# Autodesk Inventor assembly: SR-092-DPY(F,D-166-1)
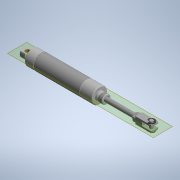
[picture p0: Inventor's stored thumbnail of the model, 180x180]
Saved by Autodesk Inventor 2020 (Build 240168000, 168)
## iProperties
Part Number: SR-092-DPY(F,D-166-1)
Catalog Web Link: www.cadenas.de
Description: Original Line Standard Air Cylinders-Standard Air Cylinders
Vendor: BIMBA
Document SubType Name: Assembly
Designer: partserver
Manufacturer: BIMBA
Mass: 56.1668 g
Surface Area: 355.51 cm^2
Volume: 56.1668 cm^3
Density: 1 g/cm^3
Category: PARTsolutions
Company: BIMBA
PSOL_IDENT_0: {$CADENAS_DATA\23d-libs\bimba\bimba_brand\bimba_imperial\bimba_full_line\original_line_cylinders\sta
PSOL_IDENT_1: ndard_air_cylinders\standard_air_cylinder_asmtab.prj},348 {VTYP=3D},{STYP=ASSTAB},{NB=SR-092-DPY(F,D
PSOL_IDENT_2: -166-1)},{LINA=SR-092-DPY(D-166-1)},{NN=Original Line Standard Air Cylinders},{DATE=19.01.2022 10:19
PSOL_IDENT_3: :38},{GEOMDATE=11.11.2021 07:31:43},{VERSION=},{LINEID=10},{WBVAR=STROKE,ACTING,MNT,DER,NR,BM,CO,OO,
PSOL_IDENT_4: VO,M,EE,EEL,K,Q,Y,G,T,HL,B,H,SER,SR,NT,W,STPT1,STPT2,STPT3,STPT4,MB,PB,PRC,TB,MN},{WBNUMERIC=STROKE,
PSOL_IDENT_5: EEL}  {NB=SR-092-DPY(F,D-166-1)},{LINA=SR-092-DPY(D-166-1)},{KT=DUMMY},{PN=SR-092-DPY},{PNC=SR-092-D
PSOL_IDENT_6: PY(F,D-166-1)},{PNA=(D-166-1)},{PNAHELP=(D-166-1)},{DASH=-},{BORE1=1.06250000},{BORE=1 1/16\" (09)},
PSOL_IDENT_7: {BOREPN=09},{STROKE=2.000},{STROKEALG=[0.011:50/0.001]},{STROKE1=2.000},{ACTING=D},{ACTINGALG= '' , '
PSOL_IDENT_8: Single Acting' , 'R' , 'Reverse Single Acting (R)' , 'D' , 'Double Acting (D)' },{ACTINGPN=D},{MNT=P
PSOL_IDENT_9: },{MNTALG= '' , 'Front Nose Mounting' , 'P' , 'Rear Pivot Mounting (P)' , 'X' , 'Universal Pivot Mou
PSOL_IDENT_10: nting or Double End Mounting (X)' , 'BF' , 'Front Block Mounting (BF)' , 'BR' , 'Rear Block Mounting
PSOL_IDENT_11: for Vertical Positioning (BR)' , 'BFT' , 'Front Block Trunnion Mounting (BFT)' , 'BRT' , 'Rear Bloc
PSOL_IDENT_12: k Trunnion Mounting (BRT)' },{TYPE=SR-},{MNTPN=P},{DER=},{DERALG= '' , 'N/A' },{NR=},{NRALG= '' , 'N
PSOL_IDENT_13: /A' },{NRPN=},{BM=},{BMALG= '' , 'N/A' },{BMPN=},{CO=},{COALG= '' , 'N/A' },{OO=},{OOALG= '', 'N/A'
PSOL_IDENT_14: },{OOPN=},{VO=Z},{VOALG= 'Z' , 'N/A' },{VOPN=},{OOVOPN=},{M=},{MALG= '', 'Without Magnet', 'M', 'Wit
PSOL_IDENT_15: h Magnet' },{EE=},{EEL=0.000},{EEMAX=48.0000},{EEALG= '', 'Without Extra Extension', 'EE', 'With Ext
PSOL_IDENT_16: ra Extension' },{EELALG=0},{EEPN=},{EEPN1=0.000},{K=},{KALG= '', 'Standard' , 'K' , 'Ports Rotated 9
PSOL_IDENT_17: 0deg K' },{KPN=},{Q=},{QALG= '' , 'N/A' },{QPN=},{Y=Y},{YALG= '' , 'Without Pivot Bushing' , 'Y' , '
PSOL_IDENT_18: With Pivot Bushing' },{YPN=Y},{YCON=Y},{F=},{FALG= '', 'Non-Coated (Standard)', 'F', 'Molycoated' },
PSOL_IDENT_19: {FPN=},{G=},{GPN=},{GPN99=},{T=},{TALG= '' , 'Standard -20° to 200°F (-29° to 95°C)' , 'N' , 'Low Te
PSOL_IDENT_20: mperature' , 'V' , 'High Temperature' },{NPN=},{VPN=},{HL=},{HLALG= '' , 'Without Low Pressure Hydra
PSOL_IDENT_21: ulic' , 'HL' , 'With Low Pressure Hydraulic' },{B=},{BALG= '', 'W/out Bumpers' , 'B' , 'W/ Bumpers'
PSOL_IDENT_22: },{BPN=},{H=},{HALG= '', 'N/A' },{HPN=},{SER=},{SERALG= '' , 'Without Spring Extend/Return' , 'JS' ,
PSOL_IDENT_23: 'With Spring Return' , 'JR' , 'With Spring Extend' },{SR=SR},{SRALG= 'C' , 'Standard Blackened Carb
PSOL_IDENT_24: on Steel' , 'SR' , 'Stainless Steel [SR]' },{SRPN=SR},{SRCON=1},{NT=},{NTPN=},{W=},{WALG= '' , 'With
PSOL_IDENT_25: out Wiper' , 'W' , 'With Wiper' },{WPN=},{E=},{EALG= '' , 'Standard Seals/Lube' , 'E' , 'Non-Lube Se
PSOL_IDENT_26: als/Lube' },{EPN=},{ST=},{STALG= '' , 'N/A' },{STPT1=},{STPT1ALG= '' , 'N/A' },{STPT2=},{STPT2ALG= ''
PSOL_IDENT_27: , 'N/A' },{STPT3=},{STPT3ALG= '' , 'N/A' },{STPT4=},{STPT4ALG= '' , 'N/A' },{STPN=},{MB=},{MBALG= ''
PSOL_IDENT_28: , 'N/A' },{MBPN=},{MBPNALL=},{MBPNALLREAR=},{PB=},{PBALG= '' , 'Without Pivot Bracket' , 'D-13498-A'
PSOL_IDENT_29: , 'D-13498-A' },{PBPN=},{PBPNALL=D-13498-A},{PRC=F,D-166-1},{PRCALG= '' , 'W/out Pivot Rod Clevis'
PSOL_IDENT_30: , 'F,D-166-1' , 'D-166-1 (front)' },{PRCPN=(F,D-166-1)},{PRCPNALL=D-166-1},{TB=},{TBALG= '' , 'N/A'
PSOL_IDENT_31: },{TBPN=},{TBPNALL=},{MN=},{MNALG= '' , 'Without Mounting Nut' , 'F,D-9' , 'D-9 (front)' , 'R,D-9' ,
PSOL_IDENT_32: 'D-9 (rear)', '2x,D-9' , 'D-9 (front & rear)' },{MNPN=},{MNCONF=},{MNCONR=},{TLEN=3.3185},{FRAC=8.8
PSOL_IDENT_33: 400},{RGCON=},{RGDACCON=R},{RHCON=P},{RHCON1=P},{RHCONON=1},{RHACCON=},{FNUTCON=0},{RNUTCON=0},{FNUT
PSOL_IDENT_34: PN=D-9},{RNUTPN=D-9},{FNUTTRANS=0.0000},{RNUTTRANS=0.0000},{VHOLECON=0},{A1=1.6250},{A1N=1.0000},{A1
PSOL_IDENT_35: P=1.6250},{A1B=1.8750},{A4=0.2525},{A4N=0.3750},{A4P=0.2525},{A5=0.0300},{A1H=1.5},{A1NH=0.6250},{A1
PSOL_IDENT_36: PH=1.5000},{A1BH=1.1250},{A1SH=1.1250},{A2H=0.2500},{A2NH=0.2500},{LENGTH=3.8400},{LENGTH1=3.8400},{
PSOL_IDENT_37: LENGTH2=4.1000},{MUL=2.0000},{MUL11=2.0000},{MUL22=5.12},{MUL33=3.1200},{MUL2=2.0000},{MUL211=2.0000
PSOL_IDENT_38: },{MUL222=2.5600},{MUL233=1.5600},{SSS=4.0000},{RGLEN=1.4025},{RHLEN=0.9990},{SSS1=3.0000},{A13=1.21
PSOL_IDENT_39: 90},{DIF=0.1200},{G5=0.7180},{ON=0},{SSADD=0.0000},{BADD=0.0000},{MADD=0.0000},{NVADD=0.0000},{TRACK
PSOL_IDENT_40: L=3.0285},{TRACKCON=D-78527},{TRIMCON=0},{TRIMCON1=0},{PINCON=},{FSPACE=0.7526},{SPACE=0.0911},{TEXT=
PSOL_IDENT_41: 0.1594},{S1=1.2500},{D1=1.1410},{D1N=1.1130},{D1B=1.1130},{D1P=1.1410},{FA=0.940},{RA=0.9400},{PPATH=
PSOL_IDENT_42: standard_air_cylinder_asmtpl.prj},{MATALGHTML=<b>Standard Original Line:</b><dl><dt>Rod:</dt><dd>- S
PSOL_IDENT_43: tainless Steel</dd><dd>&nbsp;&nbsp;(5/16 9/16 Bores)</dd><dd>- High Strength Carbon Steel</dd><dd>&n
PSOL_IDENT_44: bsp;&nbsp;(3/4 3 Bore)</dd><dd>- Stainless Steel</dd><dd>&nbsp;&nbsp;(X style DXP/DX/DXDE)</dd><dt>B
PSOL_IDENT_45: earings:</dt><dd>- Sintered Bronze</dd><dt>Body:</dt><dd>- 304 Stainless Steel</dd><dt>End Caps:</dt
PSOL_IDENT_46: ><dd>- Aluminum</dd><dt>Seals:</dt><dd>- Buna N</dd></dl>},{ASSCFGPRA=09DP},{MBPNA=},{MNPNA=},{PRCPN
PSOL_IDENT_47: A=(D-166-1)},{ASSOPTACC=STPT4},{A=5.84},{HADD=0.0000},{WFL=0.125},{QADD=0.000},{QADD1=0.250},{TEST=2
PSOL_IDENT_48: .0000},{MNTB=},{STDNUTF=0},{STDNUTR=0},{STRK2D=0},{X2D=2},{STROKESW=2.000},{EESW=0.000},{FCD=0},{BCD=
PSOL_IDENT_49: 0},{RCD=0},{CUSTADD=1.000},{FT=5/16-24 UNF-2A},{FT1=5/16-24 UNF-2A},{FT2=5/8-18 UNF-2A},{PORT=1/8 NP
PSOL_IDENT_50: T},{FT11=5/8-18 UNF-2A},{FT12=5/8-18 UNF-2A},{B1=}
NB: SR-092-DPY(F,D-166-1)
NN: Original Line Standard Air Cylinders
NT: Threaded (Standard)
NBSYN: $PNC.
LINA: SR-092-DPY(D-166-1)
CATALOG: Bimba Products
PN: SR-092-DPY
PNA: (D-166-1)
BORE: 1 1/16" (09)
STROKE: 2
ACTING: Double Acting (D)
MNT: Rear Pivot Mounting (P)
DER: N/A
NR: N/A
BM: N/A
CO: N/A
OO: N/A
VO: N/A
M: Without Magnet
EE: Without Extra Extension
EEL: 0
K: Standard
Q: N/A
Y: With Pivot Bushing
G: Standard Lube
T: Standard -20° to 200°F (-29° to 95°C)
HL: Without Low Pressure Hydraulic
B: W/out Bumpers
H: N/A
SER: Without Spring Extend/Return
SR: Stainless Steel [SR]
W: Without Wiper
STPT1: N/A
STPT2: N/A
STPT3: N/A
STPT4: N/A
MB: N/A
PB: Without Pivot Bracket
PRC: D-166-1 (front)
TB: N/A
MN: Without Mounting Nut
A: 5.84
SUPPLIER: BIMBA
ARTICLENO: SR-092-DPY(F,D-166-1)
BOMINFO: SR-092-DPY(D-166-1)
CREATOR: CADENAS GmbH
Title: SR-092-DPY(D-166-1)
Author: Cadenas PARTsolutions
Comments: Standard Air Cylinders
## Documents named in this file (12)
- T:\EIT\2022 Rapid React\COMMON PARTS\AIR CYLINDERS\BIMBA_SR092DPYFD1661\AIS2020\SR-092-DPY(F,D-166-1).iam
- T:\EIT\2022 Rapid React\COMMON PARTS\AIR CYLINDERS\BIMBA_SR092DPYFD1661\AIS2020\SR-092-DPSRY(F,D-166-1)0000000_0_dummy.ipt
- T:\EIT\2022 Rapid React\COMMON PARTS\AIR CYLINDERS\BIMBA_SR092DPYFD1661\AIS2020\09R000-0_rod_guide.ipt
- T:\EIT\2022 Rapid React\COMMON PARTS\AIR CYLINDERS\BIMBA_SR092DPYFD1661\AIS2020\09R-3_31350SR.ipt
- T:\EIT\2022 Rapid React\COMMON PARTS\AIR CYLINDERS\BIMBA_SR092DPYFD1661\AIS2020\09P0Y000_rear_head.ipt
- T:\EIT\2022 Rapid React\COMMON PARTS\AIR CYLINDERS\BIMBA_SR092DPYFD1661\AIS2020\D-3543.ipt
- T:\EIT\2022 Rapid React\COMMON PARTS\AIR CYLINDERS\BIMBA_SR092DPYFD1661\AIS2020\SR-092-DPY0000_rod.ipt
- T:\EIT\2022 Rapid React\COMMON PARTS\AIR CYLINDERS\BIMBA_SR092DPYFD1661\AIS2020\D-166-1-dummy.ipt
- T:\EIT\2022 Rapid React\COMMON PARTS\AIR CYLINDERS\BIMBA_SR092DPYFD1661\AIS2020\D-14059.ipt
- T:\EIT\2022 Rapid React\COMMON PARTS\AIR CYLINDERS\BIMBA_SR092DPYFD1661\AIS2020\D-8381.ipt
- T:\EIT\2022 Rapid React\COMMON PARTS\AIR CYLINDERS\BIMBA_SR092DPYFD1661\AIS2020\D-5866.ipt
- T:\EIT\2022 Rapid React\COMMON PARTS\AIR CYLINDERS\BIMBA_SR092DPYFD1661\AIS2020\D-746.ipt
## Components (12 placed, 11 different names)
1. SR-092-DPSRY(F,D-166-1)0000000_0_dummy:1
2. 09R000-0_rod_guide:1
3. 09R-3_31350SR:1
4. 09P0Y000_rear_head:1 — Insert:6, Angle:1
5. D-3543:1
6. SR-092-DPY0000_rod:1 — Insert:3, Insert:6
7. D-166-1-dummy:1
8. D-14059:1 — Insert:4, Angle:1, Insert:7
9. D-8381:1 — Insert:1, Insert:2
10. D-5866:1 — Insert:1
11. D-5866:2 — Insert:2, Insert:7
12. D-746:1 — Insert:3, Insert:4
## Relationships (7: Insert 6, Angle 1)
- Insert:1: D-8381:1 ↔ D-5866:1
- Insert:2: D-8381:1 ↔ D-5866:2
- Insert:3: SR-092-DPY0000_rod:1 ↔ D-746:1
- Insert:4: D-14059:1 ↔ D-746:1
- Insert:6: 09P0Y000_rear_head:1 ↔ SR-092-DPY0000_rod:1
- Angle:1 (0 deg): 09P0Y000_rear_head:1 ↔ D-14059:1
- Insert:7: D-14059:1 ↔ D-5866:2
